# Autodesk Inventor assembly: cycloid_reducer
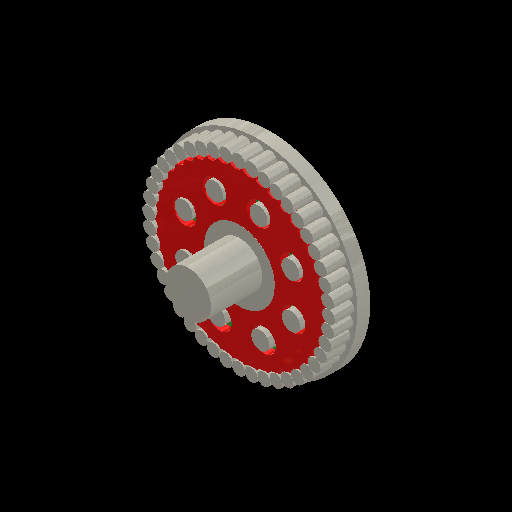
[picture p0: Inventor's stored thumbnail of the model, 512x512]
Saved by Autodesk Inventor 2026 (Build 300175050, 175E)
## iProperties
Created: 2026-06-07
Part Number: cycloid_reducer
Document SubType Name: Assembly
Designer: iamma
Author: iamma
## Documents named in this file (5)
- C:\Users\iamma\OneDrive\바탕 화면\LEE\2026-1\최적설계\Optimum_Design_Proj\사이클로이드 감속기\OptimumDesign_CycloidReducer\3d_model\cycloid_reducer.iam
- C:\Users\iamma\OneDrive\바탕 화면\LEE\2026-1\최적설계\Optimum_Design_Proj\사이클로이드 감속기\OptimumDesign_CycloidReducer\3d_model\housing.ipt
- C:\Users\iamma\OneDrive\바탕 화면\LEE\2026-1\최적설계\Optimum_Design_Proj\사이클로이드 감속기\OptimumDesign_CycloidReducer\3d_model\input_shaft.ipt
- C:\Users\iamma\OneDrive\바탕 화면\LEE\2026-1\최적설계\Optimum_Design_Proj\사이클로이드 감속기\OptimumDesign_CycloidReducer\3d_model\cycloid_gear.ipt
- C:\Users\iamma\OneDrive\바탕 화면\LEE\2026-1\최적설계\Optimum_Design_Proj\사이클로이드 감속기\OptimumDesign_CycloidReducer\3d_model\out_shaft.ipt
## Components (5 placed, 4 different names)
1. housing:1 — 메이트:1, 메이트:2, 각도:1, 각도:2, 각도:3, 메이트:5, 플러쉬:3, 각도:4
2. input_shaft:1 — 메이트:1, 메이트:2, 메이트:3, 플러쉬:1, 메이트:4, 플러쉬:2, 각도:1
3. cycloid_gear:1 — 메이트:3, 플러쉬:1, 각도:2
4. cycloid_gear:2 — 메이트:4, 플러쉬:2, 각도:3
5. out_shaft:1 — 메이트:5, 플러쉬:3, 각도:4
## Relationships (12: Mate 5, Angle 4, Flush 3)
- 메이트:1 [Mate]: housing:1 ↔ input_shaft:1
- 메이트:2 [Mate]: housing:1 ↔ input_shaft:1
- 메이트:3 [Mate]: input_shaft:1 ↔ cycloid_gear:1
- 플러쉬:1 [Flush]: input_shaft:1 ↔ cycloid_gear:1
- 메이트:4 [Mate]: input_shaft:1 ↔ cycloid_gear:2
- 플러쉬:2 [Flush]: input_shaft:1 ↔ cycloid_gear:2
- 각도:1 [Angle] (915 deg): housing:1 ↔ input_shaft:1
- 각도:2 [Angle] (-21.2791 deg): housing:1 ↔ cycloid_gear:1
- 각도:3 [Angle] (-25.4651 deg): housing:1 ↔ cycloid_gear:2
- 메이트:5 [Mate]: housing:1 ↔ out_shaft:1
- 플러쉬:3 [Flush] (-2 mm): housing:1 ↔ out_shaft:1
- 각도:4 [Angle] (-23.3721 deg): housing:1 ↔ out_shaft:1
